# Autodesk Inventor assembly: 頭
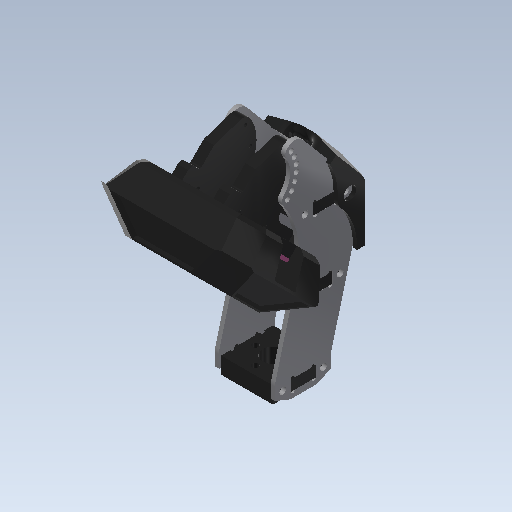
[picture p0: Inventor's stored thumbnail of the model, 512x512]
Saved by Autodesk Inventor 2020 (Build 240168000, 168)
## iProperties
Created: 2018-06-08
Part Number: 頭
Material: 一般
Document SubType Name: Assembly
Designer: taka
Mass: 93.8515 g
Surface Area: 499.568 cm^2
Volume: 83.6319 cm^3
Density: 1.1222 g/cm^3
Author: taka
## Documents named in this file (9)
- C:\Users\6343y\Documents\Inventor\GankenKun\OpenPlatform_ver3_0\上半身\頭\頭.iam
- C:\Users\6343y\Documents\Inventor\GankenKun\OpenPlatform_ver3_0\上半身\頭\頭_メインフレーム.ipt
- C:\Users\6343y\Documents\Inventor\GankenKun\OpenPlatform_ver3_0\上半身\頭\頭_サブフレーム.ipt
- C:\Users\6343y\Documents\Inventor\GankenKun\OpenPlatform_ver3_0\上半身\頭\頭_サーボホーンフレーム.ipt
- C:\Users\6343y\Documents\Inventor\GankenKun\OpenPlatform_ver3_0\上半身\頭\カメラ_メインフレーム.ipt
- C:\Users\6343y\Documents\Inventor\GankenKun\OpenPlatform_ver3_0\上半身\頭\カメラ_メインフレーム1_KBCR-S02MU.ipt
- C:\Users\6343y\Documents\Inventor\GankenKun\OpenPlatform_ver3_0\上半身\頭\KBCR-S02MU.ipt
- C:\Users\6343y\Documents\Inventor\GankenKun\OpenPlatform_ver3_0\上半身\頭\カメラ_外装.ipt
- C:\Users\6343y\Documents\Inventor\GankenKun\OpenPlatform_ver3_0\上半身\頭\CameraCable_Assist.ipt
## Components (11 placed, 8 different names)
1. 頭_メインフレーム:1 — 挿入:1, 挿入:5, 挿入:6, 挿入:8, 挿入:22, 挿入:23, 挿入:29
2. 頭_メインフレーム:2 — 挿入:2, 挿入:3, 挿入:4, 挿入:7, 挿入:17, 挿入:18, 角度:1
3. 頭_サブフレーム:1 — 挿入:1, 挿入:2, 挿入:4
4. 頭_サブフレーム:2 — 挿入:3, 挿入:5, 挿入:6
5. 頭_サーボホーンフレーム:1 — 挿入:7, 挿入:8
6. カメラ_メインフレーム:1 — 挿入:22, 挿入:23, 挿入:25
7. カメラ_メインフレーム:2 — 挿入:17, 挿入:18, 挿入:24
8. カメラ_メインフレーム1_KBCR-S02MU:1 — 挿入:24, 挿入:25, 挿入:26, 挿入:27, 挿入:28, 正接:1
9. KBCR-S02MU:1 — 挿入:26, 挿入:27
10. カメラ_外装:1 — 挿入:28, 正接:1
11. CameraCable_Assist:1 — 挿入:29, 角度:1
## Relationships (20: Insert 18, Tangent 1, Angle 1)
- 挿入:1 [Insert]: 頭_メインフレーム:1 ↔ 頭_サブフレーム:1
- 挿入:2 [Insert]: 頭_メインフレーム:2 ↔ 頭_サブフレーム:1
- 挿入:3 [Insert]: 頭_メインフレーム:2 ↔ 頭_サブフレーム:2
- 挿入:4 [Insert]: 頭_メインフレーム:2 ↔ 頭_サブフレーム:1
- 挿入:5 [Insert]: 頭_メインフレーム:1 ↔ 頭_サブフレーム:2
- 挿入:6 [Insert]: 頭_メインフレーム:1 ↔ 頭_サブフレーム:2
- 挿入:7 [Insert]: 頭_メインフレーム:2 ↔ 頭_サーボホーンフレーム:1
- 挿入:8 [Insert]: 頭_メインフレーム:1 ↔ 頭_サーボホーンフレーム:1
- 挿入:17 [Insert]: 頭_メインフレーム:2 ↔ カメラ_メインフレーム:2
- 挿入:18 [Insert]: 頭_メインフレーム:2 ↔ カメラ_メインフレーム:2
- 挿入:22 [Insert]: 頭_メインフレーム:1 ↔ カメラ_メインフレーム:1
- 挿入:23 [Insert]: 頭_メインフレーム:1 ↔ カメラ_メインフレーム:1
- 挿入:24 [Insert]: カメラ_メインフレーム:2 ↔ カメラ_メインフレーム1_KBCR-S02MU:1
- 挿入:25 [Insert]: カメラ_メインフレーム:1 ↔ カメラ_メインフレーム1_KBCR-S02MU:1
- 挿入:26 [Insert]: カメラ_メインフレーム1_KBCR-S02MU:1 ↔ KBCR-S02MU:1
- 挿入:27 [Insert]: カメラ_メインフレーム1_KBCR-S02MU:1 ↔ KBCR-S02MU:1
- 挿入:28 [Insert]: カメラ_メインフレーム1_KBCR-S02MU:1 ↔ カメラ_外装:1
- 正接:1 [Tangent]: カメラ_メインフレーム1_KBCR-S02MU:1 ↔ カメラ_外装:1
- 挿入:29 [Insert]: 頭_メインフレーム:1 ↔ CameraCable_Assist:1
- 角度:1 [Angle] (180 deg): 頭_メインフレーム:2 ↔ CameraCable_Assist:1
